# Autodesk Inventor assembly: ASY ДМФ 030 кольцо со шпильками корма
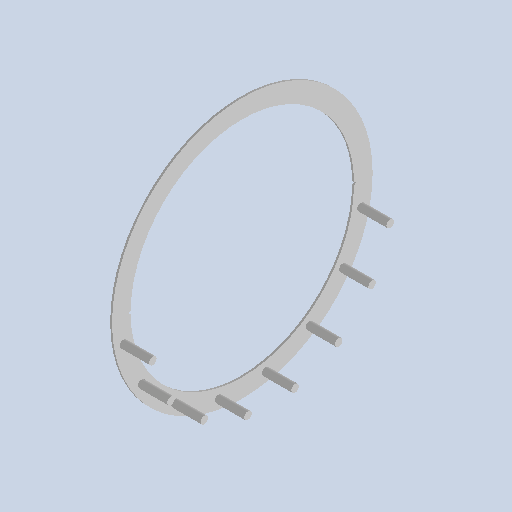
[picture p0: Inventor's stored thumbnail of the model, 512x512]
Saved by Autodesk Inventor 2025 (Build 290162010, 162A)
## iProperties
Created: 2024-04-23
Part Number: ASY ДМФ 030 кольцо со шпильками корма
Document SubType Name: Assembly
Designer: admin
Author: admin
## Documents named in this file (4)
- C:\Users\pokla\Documents\Inventor\ДФО\ДМФ\DMF-Disk-Micro-Filter\DMF old version\ASY ДМФ 030 кольцо со шпильками корма.iam
- C:\Users\pokla\Documents\Inventor\ДФО\ДМФ\DMF-Disk-Micro-Filter\DMF old version\ДМФ 031 кольцо под шпильки НОС.ipt
- C:\Users\pokla\Documents\Inventor\ДФО\ДМФ\DMF-Disk-Micro-Filter\DMF old version\ДМФ 000 размеры.ipt
- C:\Users\pokla\Documents\Inventor\ДФО\ДМФ\DMF-Disk-Micro-Filter\DMF old version\ДМС 033 шпилька 3.ipt
## Components (9 placed, 2 different names)
1. ДМФ 031 кольцо под шпильки НОС.ipt:1 — Mate:1, Rigid:1
2. ДМС 033 шпилька 3.ipt:1 — Rigid:1
3. ДМС 033 шпилька 3.ipt:2
4. ДМС 033 шпилька 3.ipt:3
5. ДМС 033 шпилька 3.ipt:4
6. ДМС 033 шпилька 3.ipt:5
7. ДМС 033 шпилька 3.ipt:6
8. ДМС 033 шпилька 3.ipt:7
9. ДМС 033 шпилька 3.ipt:8
## Component patterns: (8 elements, first: ДМС 033 шпилька 3.ipt:1)
## Relationships (2: Mate 1, WeldJoint 1)
- Mate:1: ДМФ 031 кольцо под шпильки НОС.ipt:1
- Rigid:1 [WeldJoint]: ДМФ 031 кольцо под шпильки НОС.ipt:1 ↔ ДМС 033 шпилька 3.ipt:1
